# Autodesk Inventor assembly: Wrist_B
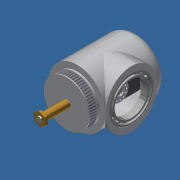
[picture p0: Inventor's stored thumbnail of the model, 180x180]
Saved by Autodesk Inventor 2016 (Build 200138000, 138)
## iProperties
Created: 2015-09-09
Part Number: Wrist_B
Material: Generisch
Document SubType Name: Assembly
Designer: 4ndreas
Mass: 222.236 g
Surface Area: 593.048 cm^2
Volume: 155.585 cm^3
Density: 1.42839 g/cm^3
Author: 4ndreas
## Documents named in this file (10)
- C:\Users\4ndreas\Documents\Inventor\RobotARM v2\v4\Wrist_B.iam
- C:\Users\4ndreas\Documents\Inventor\Content Center Files\R2014\de-DE\DIN BEARING(1)\DIN 625 SKF - SKF 61807.ipt
- C:\Users\4ndreas\Documents\Inventor\RobotARM v2\v4\60zGelenk.ipt
- C:\Users\4ndreas\Documents\Inventor\RobotARM v2\v4\[HerkuleX] DRS-010X.iam
- C:\Users\4ndreas\Documents\Inventor\Content Center Files\R2014\de-DE\DIN 912\DIN 912 - M2 x 0,4 x 20 x 19.ipt
- C:\Users\4ndreas\Documents\Inventor\RobotARM v2\v4\Bolzen.ipt
- C:\Users\4ndreas\Documents\Inventor\RobotARM v2\v4\Wrist_Cover.ipt
- C:\Users\4ndreas\Documents\Inventor\Content Center Files\R2014\de-DE\DIN 912\DIN 912 - M3 x 0,5 x 10 x 8,75.ipt
- C:\Users\4ndreas\Documents\Inventor\Content Center Files\R2014\de-DE\DIN 985\DIN 985 - M8.ipt
- C:\Users\4ndreas\Documents\Inventor\RobotARM v2\v4\EncoderMagnet.ipt
## Components (15 placed, 9 different names)
1. 60zGelenk:1 — Passend:1, Passend:2, Passend:3, Fluchtend:1, Fluchtend:2, Fluchtend:3, Passend:8, Passend:9, Passend:10, Passend:11, Passend:12, Passend:13, Passend:14, Passend:15, Passend:16, Passend:17, Passend:18, Passend:19, Passend:21, Fluchtend:4, Passend:29, Passend:30, Passend:31, Passend:33, Passend:34, Passend:36, Winkel:2, Passend:38, Passend:39
2. DIN 625 SKF SKF 61807:1 — Passend:1, Passend:2, Passend:4, Passend:29, Passend:30
3. [HerkuleX] DRS-010X:1 [sub-assembly] — Passend:5, Fluchtend:1, Winkel:1
4. DIN 912 - ersetzt durch DIN EN ISO 4762 M2 x 20:1 — Passend:8, Passend:19
5. DIN 912 - ersetzt durch DIN EN ISO 4762 M2 x 20:2 — Passend:9, Passend:18
6. DIN 912 - ersetzt durch DIN EN ISO 4762 M2 x 20:3 — Passend:10, Passend:17
7. DIN 912 - ersetzt durch DIN EN ISO 4762 M2 x 20:4 — Passend:11, Passend:14
8. DIN 912 - ersetzt durch DIN EN ISO 4762 M2 x 20:5 — Passend:13, Passend:16
9. DIN 912 - ersetzt durch DIN EN ISO 4762 M2 x 20:6 — Passend:12, Passend:15
10. Bolzen:1 — Passend:20, Passend:21, Passend:31, Passend:37, Passend:41
11. DIN 985 - ersetzt durch DIN EN ISO 10511 M8:1 — Passend:37, Passend:38, Passend:39
12. Wrist_Cover:1 — Fluchtend:4, Passend:25, Passend:26, Passend:27, Passend:28
13. DIN 912 - ersetzt durch DIN EN ISO 4762 M3 x 10:1 — Passend:26, Passend:27, Passend:33
14. DIN 912 - ersetzt durch DIN EN ISO 4762 M3 x 10:2 — Passend:25, Passend:28, Passend:34
15. EncoderMagnet:1 — Passend:40, Passend:41
## Relationships (41: Mate 35, Flush 4, Angle 2)
- Passend:1 [Mate]: 60zGelenk:1 ↔ DIN 625 SKF SKF 61807:1
- Passend:2 [Mate]: 60zGelenk:1 ↔ DIN 625 SKF SKF 61807:1
- Passend:3 [Mate]: 60zGelenk:1
- Passend:4 [Mate]: DIN 625 SKF SKF 61807:1
- Passend:5 [Mate]: [HerkuleX] DRS-010X:1
- Fluchtend:1 [Flush] (5 mm): 60zGelenk:1 ↔ [HerkuleX] DRS-010X:1
- Fluchtend:2 [Flush]: 60zGelenk:1
- Winkel:1 [Angle] (90 deg): [HerkuleX] DRS-010X:1
- Fluchtend:3 [Flush]: 60zGelenk:1
- Passend:8 [Mate]: 60zGelenk:1 ↔ DIN 912 - ersetzt durch DIN EN ISO 4762 M2 x 20:1
- Passend:9 [Mate]: 60zGelenk:1 ↔ DIN 912 - ersetzt durch DIN EN ISO 4762 M2 x 20:2
- Passend:10 [Mate]: 60zGelenk:1 ↔ DIN 912 - ersetzt durch DIN EN ISO 4762 M2 x 20:3
- Passend:11 [Mate]: 60zGelenk:1 ↔ DIN 912 - ersetzt durch DIN EN ISO 4762 M2 x 20:4
- Passend:12 [Mate]: 60zGelenk:1 ↔ DIN 912 - ersetzt durch DIN EN ISO 4762 M2 x 20:6
- Passend:13 [Mate]: 60zGelenk:1 ↔ DIN 912 - ersetzt durch DIN EN ISO 4762 M2 x 20:5
- Passend:14 [Mate]: 60zGelenk:1 ↔ DIN 912 - ersetzt durch DIN EN ISO 4762 M2 x 20:4
- Passend:15 [Mate]: 60zGelenk:1 ↔ DIN 912 - ersetzt durch DIN EN ISO 4762 M2 x 20:6
- Passend:16 [Mate]: 60zGelenk:1 ↔ DIN 912 - ersetzt durch DIN EN ISO 4762 M2 x 20:5
- Passend:17 [Mate]: 60zGelenk:1 ↔ DIN 912 - ersetzt durch DIN EN ISO 4762 M2 x 20:3
- Passend:18 [Mate]: 60zGelenk:1 ↔ DIN 912 - ersetzt durch DIN EN ISO 4762 M2 x 20:2
- Passend:19 [Mate]: 60zGelenk:1 ↔ DIN 912 - ersetzt durch DIN EN ISO 4762 M2 x 20:1
- Passend:20 [Mate]: Bolzen:1
- Passend:21 [Mate] (26 mm): 60zGelenk:1 ↔ Bolzen:1
- Fluchtend:4 [Flush]: 60zGelenk:1 ↔ Wrist_Cover:1
- Passend:25 [Mate]: Wrist_Cover:1 ↔ DIN 912 - ersetzt durch DIN EN ISO 4762 M3 x 10:2
- Passend:26 [Mate]: Wrist_Cover:1 ↔ DIN 912 - ersetzt durch DIN EN ISO 4762 M3 x 10:1
- Passend:27 [Mate]: Wrist_Cover:1 ↔ DIN 912 - ersetzt durch DIN EN ISO 4762 M3 x 10:1
- Passend:28 [Mate]: Wrist_Cover:1 ↔ DIN 912 - ersetzt durch DIN EN ISO 4762 M3 x 10:2
- Passend:29 [Mate]: 60zGelenk:1 ↔ DIN 625 SKF SKF 61807:1
- Passend:30 [Mate]: 60zGelenk:1 ↔ DIN 625 SKF SKF 61807:1
- Passend:31 [Mate]: 60zGelenk:1 ↔ Bolzen:1
- Passend:33 [Mate]: 60zGelenk:1 ↔ DIN 912 - ersetzt durch DIN EN ISO 4762 M3 x 10:1
- Passend:34 [Mate]: 60zGelenk:1 ↔ DIN 912 - ersetzt durch DIN EN ISO 4762 M3 x 10:2
- Passend:35 [Mate]
- Passend:36 [Mate]: 60zGelenk:1
- Winkel:2 [Angle] (0 deg): 60zGelenk:1
- Passend:37 [Mate]: Bolzen:1 ↔ DIN 985 - ersetzt durch DIN EN ISO 10511 M8:1
- Passend:38 [Mate]: 60zGelenk:1 ↔ DIN 985 - ersetzt durch DIN EN ISO 10511 M8:1
- Passend:39 [Mate]: 60zGelenk:1 ↔ DIN 985 - ersetzt durch DIN EN ISO 10511 M8:1
- Passend:40 [Mate]: EncoderMagnet:1
- Passend:41 [Mate]: Bolzen:1 ↔ EncoderMagnet:1
